# Autodesk Inventor assembly: Mithril Cover
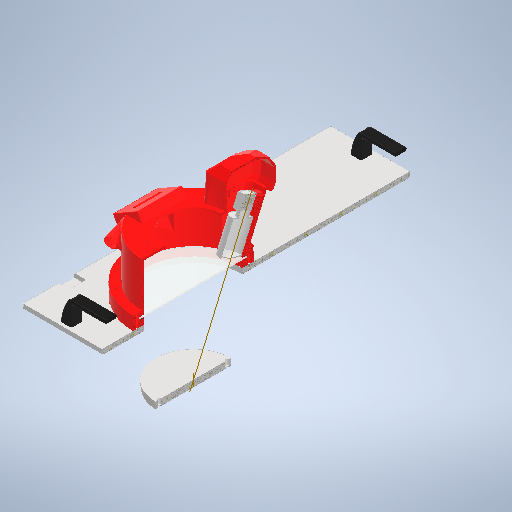
[picture p0: Inventor's stored thumbnail of the model, 512x512]
Saved by Autodesk Inventor 2026.2 (Build 302298000, 298)
## iProperties
Created: 2026-01-15
Part Number: Mithril Cover
Document SubType Name: Assembly
Designer: mumin
Author: mumin
## Documents named in this file (11)
- C:\GitHub\In-situ-monitoring-of-powder-bed-fusion-additive-manufacturing\system_development\Mithril\v0.4\hardware_design\Mithril Cover.iam
- C:\GitHub\In-situ-monitoring-of-powder-bed-fusion-additive-manufacturing\system_development\Mithril\v0.4\hardware_design\12mm Cover.ipt
- C:\GitHub\In-situ-monitoring-of-powder-bed-fusion-additive-manufacturing\system_development\Mithril\v0.4\hardware_design\Optical Housing 2-27-26.ipt
- C:\GitHub\In-situ-monitoring-of-powder-bed-fusion-additive-manufacturing\system_development\Mithril\v0.4\hardware_design\SealedGlassRing.ipt
- C:\GitHub\In-situ-monitoring-of-powder-bed-fusion-additive-manufacturing\system_development\Mithril\v0.4\hardware_design\Handle.ipt
- C:\GitHub\In-situ-monitoring-of-powder-bed-fusion-additive-manufacturing\system_development\Mithril\v0.4\hardware_design\Optical Lid.ipt
- C:\GitHub\In-situ-monitoring-of-powder-bed-fusion-additive-manufacturing\system_development\Mithril\v0.4\hardware_design\Antireflective Glass.ipt
- C:\GitHub\In-situ-monitoring-of-powder-bed-fusion-additive-manufacturing\system_development\Mithril\v0.4\hardware_design\Camera with 35mm.iam
- C:\GitHub\In-situ-monitoring-of-powder-bed-fusion-additive-manufacturing\system_development\Mithril\v0.4\hardware_design\substrate plate.ipt
- C:\GitHub\In-situ-monitoring-of-powder-bed-fusion-additive-manufacturing\system_development\Mithril\v0.4\hardware_design\RubberSeal_2.8.ipt
- C:\GitHub\In-situ-monitoring-of-powder-bed-fusion-additive-manufacturing\system_development\Mithril\v0.4\hardware_design\RubberSeal_2.5.ipt
## Components (12 placed, 10 different names)
1. 12mm Cover:1 — Insert:1, Insert:3, Insert:4, Insert:5, Insert:10, Insert:14
2. Optical Housing 2-27-26:1 — Insert:2, Mate:1, Insert:6, Mate:2, Mate:3, Mate:4, Insert:8, Insert:9, Insert:12
3. SealedGlassRing:1 — Insert:1, Insert:2, Insert:5, Insert:6, Insert:11
4. Handle:1 — Insert:3
5. Handle:2 — Insert:4
6. Optical Lid:1 — Mate:1, Mate:2, Mate:3
7. Antireflective Glass:1 — Insert:13
8. Camera with 35mm:1 [sub-assembly] — Mate:4, Insert:8, Insert:9
9. substrate plate:1 — Insert:10
10. RubberSeal_2.8:1 — Insert:11, Insert:13
11. RubberSeal_2.8:2 — Insert:12
12. RubberSeal_2.5:1 — Insert:14
## Relationships (17: Insert 13, Mate 4)
- Insert:1: 12mm Cover:1 ↔ SealedGlassRing:1
- Insert:2: Optical Housing 2-27-26:1 ↔ SealedGlassRing:1
- Insert:3: 12mm Cover:1 ↔ Handle:1
- Insert:4: 12mm Cover:1 ↔ Handle:2
- Mate:1: Optical Housing 2-27-26:1 ↔ Optical Lid:1
- Insert:5: 12mm Cover:1 ↔ SealedGlassRing:1
- Insert:6: Optical Housing 2-27-26:1 ↔ SealedGlassRing:1
- Mate:2: Optical Housing 2-27-26:1 ↔ Optical Lid:1
- Mate:3: Optical Housing 2-27-26:1 ↔ Optical Lid:1
- Mate:4: Optical Housing 2-27-26:1 ↔ Camera with 35mm:1
- Insert:8: Optical Housing 2-27-26:1 ↔ Camera with 35mm:1
- Insert:9: Optical Housing 2-27-26:1 ↔ Camera with 35mm:1
- Insert:10 (150 mm): 12mm Cover:1 ↔ substrate plate:1
- Insert:11: SealedGlassRing:1 ↔ RubberSeal_2.8:1
- Insert:12: Optical Housing 2-27-26:1 ↔ RubberSeal_2.8:2
- Insert:13 (1.3 mm): Antireflective Glass:1 ↔ RubberSeal_2.8:1
- Insert:14: 12mm Cover:1 ↔ RubberSeal_2.5:1
